# Autodesk Inventor assembly: 5x14mmBoltWasher
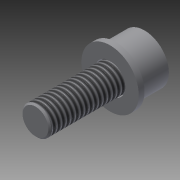
[picture p0: Inventor's stored thumbnail of the model, 180x180]
Saved by Autodesk Inventor 2014 SP1 (Build 180222100, 222)
## iProperties
Created: 2013-12-15
Part Number: 5x14mmBoltWasher
Document SubType Name: Assembly
Designer: Jack
Author: Jack
## Documents named in this file (3)
- C:\Users\Jack\Sync\MendelMax1.5\InventorParts\Hardware\BoltWashers\5x15BoltWasher.iam
- C:\Users\Jack\Sync\MendelMax1.5\InventorParts\Hardware\Bolts\M5x14SHCS.ipt
- C:\Users\Jack\Sync\MendelMax1.5\InventorParts\Hardware\Washers\M5Washer.ipt
## Components (2 placed, 2 different names)
1. M5x14SHCS:1 — Mate:1, Mate:2
2. M5Washer:1 — Mate:1, Mate:2
## Relationships (2: Mate 2)
- Mate:1: M5x14SHCS:1 ↔ M5Washer:1
- Mate:2: M5x14SHCS:1 ↔ M5Washer:1
